# Autodesk Inventor assembly: kchassis
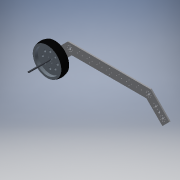
[picture p0: Inventor's stored thumbnail of the model, 180x180]
Saved by Autodesk Inventor 2016 (Build 200138000, 138)
## iProperties
Created: 2015-09-13
Part Number: kchassis
Document SubType Name: Assembly
Designer: Tim
Author: Tim
## Documents named in this file (5)
- C:\Users\Tim\Documents\GitHub\phi_robotics\3d-models\FTC_Tetrix_KOP_Block_Party\Tim Bloot Designs\kchassis.iam
- C:\Users\Tim\Documents\GitHub\phi_robotics\3d-models\FTC_Tetrix_KOP_Block_Party\Tim Bloot Designs\KrakenCsideplate1.ipt
- C:\Users\Tim\Documents\GitHub\phi_robotics\3d-models\FTC_Tetrix_KOP_Block_Party\Tetrix_Kit_FTC\Autodesk Inventor Files\tetrix_bushing.ipt
- C:\Users\Tim\Documents\GitHub\phi_robotics\3d-models\FTC_Tetrix_KOP_Block_Party\Tetrix_Kit_FTC\Autodesk Inventor Files\tetrix_axle.ipt
- C:\Users\Tim\Documents\GitHub\phi_robotics\3d-models\FTC_Tetrix_KOP_Block_Party\Tetrix_Kit_FTC\Autodesk Inventor Files\tetrix_wheel.ipt
## Components (4 placed, 4 different names)
1. KrakenCsideplate1:2 — Rotational:1
2. tetrix_bushing:1 — Rotational:1, Rotational:2, Rotational:3
3. tetrix_axle:1 — Rotational:2
4. tetrix_wheel:1 — Rotational:3
## Relationships (3: RevoluteJoint 3)
- Rotational:1 [RevoluteJoint]: KrakenCsideplate1:2 ↔ tetrix_bushing:1
- Rotational:2 [RevoluteJoint]: tetrix_bushing:1 ↔ tetrix_axle:1
- Rotational:3 [RevoluteJoint] (11 mm): tetrix_bushing:1 ↔ tetrix_wheel:1
